# Autodesk Inventor assembly: Car_Assemblage_Etudiant_2024
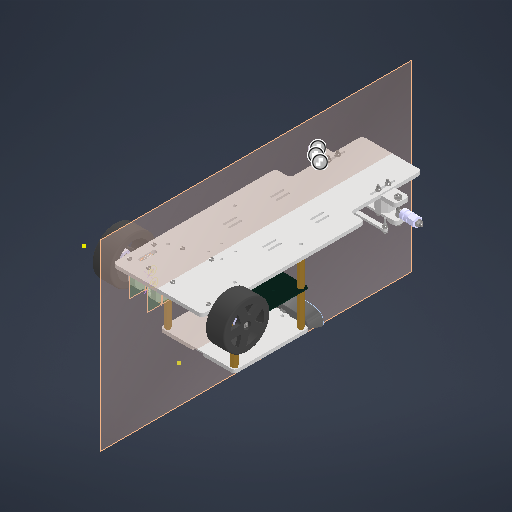
[picture p0: Inventor's stored thumbnail of the model, 512x512]
Saved by Autodesk Inventor 2027.1 (Build 311270010, 270A)
## iProperties
Created: 2023-10-18
Part Number: Car_Assemblage_Etudiant_2024
Document SubType Name: Assembly
Designer: baince
Mass: 835.359 g
Surface Area: 2295.89 cm^2
Volume: 721.463 cm^3
Density: 1.15787 g/cm^3
Author: baince
## Documents named in this file (38)
- C:\Users\thiag\Documents\ENSTA-1\Ateliers\CAO Inventor Etudiant\Car_Assemblage_Etudiant_2024.iam
- C:\Users\thiag\Documents\ENSTA-1\Ateliers\CAO Inventor Etudiant\chassis.ipt
- C:\Users\thiag\Documents\ENSTA-1\Ateliers\CAO Inventor Etudiant\support_avant.ipt
- C:\Users\thiag\Documents\ENSTA-1\Ateliers\CAO Inventor Etudiant\support_arriere_gauche.ipt
- C:\Users\thiag\Documents\ENSTA-1\Ateliers\CAO Inventor Etudiant\moteur_brushless.ipt
- C:\Users\thiag\Documents\ENSTA-1\Ateliers\CAO Inventor Etudiant\adaptateur roue.ipt
- C:\Users\thiag\Documents\ENSTA-1\Ateliers\CAO Inventor Etudiant\adaptateur_brushless.ipt
- C:\Users\thiag\Documents\ENSTA-1\Ateliers\CAO Inventor Etudiant\roue.ipt
- C:\Users\thiag\Documents\ENSTA-1\Ateliers\CAO Inventor Etudiant\biellette_servo_moteur.ipt
- C:\Users\thiag\Documents\ENSTA-1\Ateliers\CAO Inventor Etudiant\support_servo_moteur.ipt
- C:\Users\thiag\Documents\ENSTA-1\Ateliers\CAO Inventor Etudiant\SUPPORT_MOTEUR_BRUSHLESS2.IPT
- C:\Users\thiag\Documents\ENSTA-1\Ateliers\CAO Inventor Etudiant\corps_servo_moteur.ipt
- C:\Users\thiag\Documents\ENSTA-1\Ateliers\CAO Inventor Etudiant\batterie.ipt
- C:\Users\thiag\Documents\ENSTA-1\Ateliers\CAO Inventor Etudiant\roulement_6_19.ipt
- C:\Users\thiag\Documents\ENSTA-1\Ateliers\CAO Inventor Etudiant\pignon_15_dents.ipt
- C:\Users\thiag\Documents\ENSTA-1\Ateliers\CAO Inventor Etudiant\pignon_32_dents.ipt
- C:\Users\thiag\Documents\ENSTA-1\Ateliers\CAO Inventor Etudiant\axe_taraude_m4.ipt
- C:\Users\thiag\Documents\ENSTA-1\Ateliers\CAO Inventor Etudiant\roulement_4_13.ipt
- C:\Users\thiag\Documents\ENSTA-1\Ateliers\CAO Inventor Etudiant\ISO 4032 - M4 - ISO.ipt
- C:\Users\thiag\Documents\ENSTA-1\Ateliers\CAO Inventor Etudiant\ANSI B18.16.3M - Property Class 5 and 10 - Metric M3 x 0.5 Type de métal.ipt
- C:\Users\thiag\Documents\ENSTA-1\Ateliers\CAO Inventor Etudiant\ANSI B18.3.1M - M3x0,5 x 30(1).ipt
- C:\Users\thiag\Documents\ENSTA-1\Ateliers\CAO Inventor Etudiant\ISO 4762 - M4 x 30ISO.ipt
- C:\Users\thiag\Documents\ENSTA-1\Ateliers\CAO Inventor Etudiant\ISO 7089 - 4 - 140 HV(1).ipt
- C:\Users\thiag\Documents\ENSTA-1\Ateliers\CAO Inventor Etudiant\ISO 4762 - M4 x 35ISO.ipt
- C:\Users\thiag\Documents\ENSTA-1\Ateliers\CAO Inventor Etudiant\SKF623.ipt
- C:\Users\thiag\Documents\ENSTA-1\Ateliers\CAO Inventor Etudiant\ISO 7089 - 6 - 140 HV(1).ipt
- C:\Users\thiag\Documents\ENSTA-1\Ateliers\CAO Inventor Etudiant\ANSI B18.3.1M - M3x0,5 x 35(1).ipt
- C:\Users\thiag\Documents\ENSTA-1\Ateliers\CAO Inventor Etudiant\ISO 7089 - 3 - 140 HV(1).ipt
- C:\Users\thiag\Documents\ENSTA-1\Ateliers\CAO Inventor Etudiant\EN ISO 7045 - M3 x 14 - 4.8 - Z(2).ipt
- C:\Users\thiag\Documents\ENSTA-1\Ateliers\CAO Inventor Etudiant\VisM3-16.ipt
- C:\Users\thiag\Documents\ENSTA-1\Ateliers\CAO Inventor Etudiant\support_avant_MIR2.ipt
- C:\Users\thiag\Documents\ENSTA-1\Ateliers\CAO Inventor Etudiant\ESSIEU_ARRIERE.IPT
- C:\Users\thiag\Documents\ENSTA-1\Ateliers\CAO Inventor Etudiant\barre_direction.ipt
- C:\Users\thiag\Documents\ENSTA-1\Ateliers\CAO Inventor Etudiant\pcb_assembly.iam
- C:\Users\thiag\Documents\ENSTA-1\Ateliers\CAO Inventor Etudiant\sensors_haut.iam
- C:\Users\thiag\Documents\ENSTA-1\Ateliers\Seila\support_arriere_droite.ipt
- support_arriere_droite.ipt
- C:\Users\thiag\Documents\ENSTA-1\Ateliers\Seila\support_arriere_gauche_2.ipt
## Components (122 placed, 36 different names)
1. chassis:1 — Mate:1, Mate:5, Mate:19, Flush:1, Flush:2, Mate:21, Mate:22, Mate:23, Mate:26, Mate:27, Mate:28, Mate:66, Mate:68, Mate:70, Mate:72, Insert:57, Insert:58, Insert:59, Insert:60, Insert:61, Insert:62, Insert:63, Insert:64, Mate:74, Mate:75, Mate:80, Mate:102, Mate:103, Mate:104, Mate:118, Mate:120
2. ESSIEU ARRIERE:1 — Mate:115
3. support_avant:1 — Mate:1, Mate:3, Mate:4, Mate:5, Mate:7, Insert:30, Insert:84, Mate:87, Mate:89
4. moteur_brushless:1 — Mate:29, Mate:30, Mate:31, Insert:12
5. adaptateur roue:1 — Mate:43, Mate:44, Mate:45, Insert:18
6. adaptateur_brushless:1 — Mate:29, Mate:30, Mate:31, Mate:32, Mate:33, Mate:34, Insert:77, Insert:78, Insert:79, Insert:80
7. roue:1 — Mate:42, Mate:46, Mate:47, Insert:39
8. roue:2 — Mate:41, Mate:48, Mate:49, Insert:41
9. roue:3 — Mate:40, Mate:50, Mate:51, Insert:37
10. roue:4 — Mate:43, Mate:44, Mate:45, Insert:35
11. support_arriere_gauche:2 — Mate:21, Mate:22, Mate:23, Mate:36, Mate:38, Insert:65, Insert:69
12. biellette_servo_moteur:1 — Mate:15, Mate:16, Mate:101, Mate:116, Rotation:1
13. support_servo_moteur:1 — Mate:3, Mate:4, Mate:7, Mate:12, Mate:13, Mate:14, Insert:43, Insert:45, Insert:47, Insert:49, Angle:4
14. SUPPORT_MOTEUR_BRUSHLESS2:1 — Mate:26, Mate:27, Mate:28, Mate:32, Mate:33, Mate:34, Insert:66, Insert:70, Insert:73, Insert:74, Insert:75, Insert:76
15. corps_servo_moteur:1 — Mate:12, Mate:13, Mate:14, Mate:15, Mate:16
16. batterie:1 — Mate:19, Flush:1, Flush:2
17. roulement_6_19:1 — Insert:27, Mate:117
18. roulement_6_19:2 — Mate:36, Mate:38
19. adaptateur roue:2 — Mate:42, Mate:46, Mate:47
20. adaptateur roue:3 — Mate:41, Mate:48, Mate:49, Mate:115
21. adaptateur roue:4 — Mate:40, Mate:50, Mate:51, Insert:19
22. pignon_15_dents:1 — Insert:12, Tangent:1
23. pignon_32_dents:1 — Tangent:2
24. axe_taraude_m4:1 — Insert:25, Mate:63
25. roulement_4_13:1 — Insert:6, Mate:92, Mate:113
26. roulement_4_13:2 — Insert:3, Mate:114
27. roulement_4_13:3 — Insert:8, Mate:90
28. roulement_4_13:4 — Insert:10, Mate:109, Mate:110
29. ISO 4032 M4:1 — Insert:31
30. Ecrou hexagonal autofreiné - Acier Métrique Property Class 5 and 10 - Metric M3 x 0.5 Type de métal:1 — Insert:52
31. Vis à tête forgée - Métrique M3x0,5 x 30:1 — Insert:22, Mate:62
32. ISO 4762 M4 x 30:1 — Insert:2, Mate:111, Mate:112
33. ISO 4762 M4 x 30:2 — Insert:7, Mate:108, Mate:109
34. ISO 7089 4:1 — Insert:30, Insert:31
35. ISO 4762 M4 x 35:1 — Insert:83
36. ISO 4762 M4 x 35:2 — Insert:85
37. ISO 7089 4:2 — Insert:2, Insert:3
38. ISO 7089 4:3 — Insert:6, Insert:18
39. ISO 7089 4:4 — Insert:10, Insert:19
40. ISO 7089 4:5 — Insert:7, Insert:8
41. roulement_6_19:3 — Insert:25, Mate:81
42. SKF- roulements à une rangée de billes SKF623:1 — Insert:22, Insert:54
43. ISO 7089 6:1 — Insert:29, Mate:64, Mate:107
44. ISO 7089 6:2 — Insert:27
45. pignon_32_dents:2 — Mate:63, Mate:64, Tangent:1, Mate:81, Mate:107
46. pignon_15_dents:2 — Mate:62, Insert:29, Tangent:2
47. ISO 4032 M4:2 — Insert:32
48. ISO 4032 M4:3 — Insert:34
49. ISO 4032 M4:4 — Insert:36
50. ISO 4032 M4:5 — Insert:38
51. ISO 4032 M4:6 — Insert:40
52. ISO 7089 4:6 — Insert:34, Insert:35
53. ISO 7089 4:7 — Insert:36, Insert:37
54. ISO 7089 4:8 — Insert:38, Insert:39
55. ISO 7089 4:9 — Insert:40, Insert:41
56. ISO 7089 4:10 — Insert:32, Insert:96
57. Vis à tête forgée - Métrique M3x0,5 x 35:1 — Insert:42, Mate:69
58. Vis à tête forgée - Métrique M3x0,5 x 35:2 — Insert:44, Mate:71
59. Vis à tête forgée - Métrique M3x0,5 x 35:3 — Insert:48, Mate:65, Mate:76
60. Vis à tête forgée - Métrique M3x0,5 x 35:4 — Insert:46, Mate:67, Mate:79
61. Ecrou hexagonal autofreiné - Acier Métrique Property Class 5 and 10 - Metric M3 x 0.5 Type de métal:2 — Insert:50
62. Ecrou hexagonal autofreiné - Acier Métrique Property Class 5 and 10 - Metric M3 x 0.5 Type de métal:3 — Insert:51
63. Ecrou hexagonal autofreiné - Acier Métrique Property Class 5 and 10 - Metric M3 x 0.5 Type de métal:4 — Insert:53
64. ISO 7089 3:1 — Insert:44, Insert:45
65. ISO 7089 3:2 — Insert:46, Insert:47
66. ISO 7089 3:3 — Insert:52, Mate:71, Mate:72
67. ISO 7089 3:4 — Insert:53, Mate:65, Mate:66
68. ISO 7089 3:5 — Insert:48, Insert:49
69. ISO 7089 3:6 — Insert:54, Insert:55
70. ISO 7089 3:7 — Insert:50, Mate:69, Mate:70
71. ISO 7089 3:8 — Insert:42, Insert:43
72. ISO 7089 3:9 — Insert:51, Mate:67, Mate:68
73. ISO 7089 3:10 — Insert:55, Insert:56
74. ISO 7089 3:11 — Insert:56
75. NF EN ISO 7045 - Z M3 x 14 - 4.8 - Z:1 — Insert:60
76. NF EN ISO 7045 - Z M3 x 14 - 4.8 - Z:2 — Insert:59
77. NF EN ISO 7045 - Z M3 x 14 - 4.8 - Z:3 — Insert:58
78. NF EN ISO 7045 - Z M3 x 14 - 4.8 - Z:4 — Insert:57
79. NF EN ISO 7045 - Z M3 x 14 - 4.8 - Z:5 — Insert:61, Mate:123
80. NF EN ISO 7045 - Z M3 x 14 - 4.8 - Z:6 — Insert:62, Mate:119
81. NF EN ISO 7045 - Z M3 x 14 - 4.8 - Z:7 — Insert:63, Mate:122
82. NF EN ISO 7045 - Z M3 x 14 - 4.8 - Z:8 — Insert:64, Mate:121
83. Ecrou hexagonal autofreiné - Acier Métrique Property Class 5 and 10 - Metric M3 x 0.5 Type de métal:5 — Insert:65
84. Ecrou hexagonal autofreiné - Acier Métrique Property Class 5 and 10 - Metric M3 x 0.5 Type de métal:6
85. Ecrou hexagonal autofreiné - Acier Métrique Property Class 5 and 10 - Metric M3 x 0.5 Type de métal:7
86. Ecrou hexagonal autofreiné - Acier Métrique Property Class 5 and 10 - Metric M3 x 0.5 Type de métal:8 — Insert:66
87. Ecrou hexagonal autofreiné - Acier Métrique Property Class 5 and 10 - Metric M3 x 0.5 Type de métal:9 — Insert:75
88. Ecrou hexagonal autofreiné - Acier Métrique Property Class 5 and 10 - Metric M3 x 0.5 Type de métal:10 — Insert:69
89. Ecrou hexagonal autofreiné - Acier Métrique Property Class 5 and 10 - Metric M3 x 0.5 Type de métal:11 — Insert:70
90. Ecrou hexagonal autofreiné - Acier Métrique Property Class 5 and 10 - Metric M3 x 0.5 Type de métal:12 — Insert:73
91. Ecrou hexagonal autofreiné - Acier Métrique Property Class 5 and 10 - Metric M3 x 0.5 Type de métal:13
92. Ecrou hexagonal autofreiné - Acier Métrique Property Class 5 and 10 - Metric M3 x 0.5 Type de métal:14
93. Ecrou hexagonal autofreiné - Acier Métrique Property Class 5 and 10 - Metric M3 x 0.5 Type de métal:15 — Insert:74
94. Ecrou hexagonal autofreiné - Acier Métrique Property Class 5 and 10 - Metric M3 x 0.5 Type de métal:16 — Insert:76
95. NF EN ISO 7045 - Z M3 x 14 - 4.8 - Z:9 — Insert:77
96. NF EN ISO 7045 - Z M3 x 14 - 4.8 - Z:10 — Insert:78
97. NF EN ISO 7045 - Z M3 x 14 - 4.8 - Z:11 — Insert:80
98. NF EN ISO 7045 - Z M3 x 14 - 4.8 - Z:12 — Insert:79
99. VisM3-16:1 — Insert:88, Mate:126, Mate:127
100. VisM3-16:2 — Insert:89, Mate:124, Mate:125
101. Ecrou hexagonal autofreiné - Acier Métrique Property Class 5 and 10 - Metric M3 x 0.5 Type de métal:17 — Insert:87, Mate:127
102. Ecrou hexagonal autofreiné - Acier Métrique Property Class 5 and 10 - Metric M3 x 0.5 Type de métal:18 — Mate:125
103. ISO 7089 3:13
104. ISO 7089 3:14 — Insert:87
105. ISO 7089 3:15 — Insert:89, Mate:128
106. ISO 7089 4:11 — Insert:83, Insert:84
107. ISO 7089 4:12 — Insert:85, Insert:95
108. ISO 7089 3:16 — Insert:88, Mate:99
109. support_avant_MIR2:1 — Mate:74, Mate:75, Mate:76, Insert:95, Mate:79, Mate:80, Insert:96, Mate:85, Mate:88
110. barre_direction:1 — Mate:99, Mate:101, Mate:116, Mate:124, Mate:126, Rotation:1, Angle:4, Mate:128
111. ISO 7089 4:13 — Mate:88
112. ISO 7089 4:14 — Mate:85
113. ISO 7089 4:15 — Mate:87
114. ISO 7089 4:16 — Mate:89
115. ISO 7089 4:17 — Mate:91, Mate:108, Mate:110
116. ISO 7089 4:18 — Mate:90, Mate:91
117. ISO 7089 4:19 — Mate:93, Mate:111, Mate:114
118. ISO 7089 4:20 — Mate:92, Mate:93, Mate:112, Mate:113
119. pcb_assembly:1 [sub-assembly] — Mate:102, Mate:103, Mate:104, Mate:105, Mate:106
120. sensors_haut:1 [sub-assembly] — Mate:105, Mate:106
121. support_arriere_droite:1 — Mate:117, Mate:118, Mate:119, Mate:123
122. support_arriere_gauche_2:1 — Mate:120, Mate:121, Mate:122
## Relationships (173: Mate 94, Insert 70, Angle 3, Flush 2, Tangent 2, CylindricalJoint 1, RelateRotation 1)
- Mate:1: chassis:1 ↔ support_avant:1
- Mate:3: support_avant:1 ↔ support_servo_moteur:1
- Mate:4: support_avant:1 ↔ support_servo_moteur:1
- Mate:5: chassis:1 ↔ support_avant:1
- Mate:7: support_avant:1 ↔ support_servo_moteur:1
- Mate:12: support_servo_moteur:1 ↔ corps_servo_moteur:1
- Mate:13: support_servo_moteur:1 ↔ corps_servo_moteur:1
- Mate:14: support_servo_moteur:1 ↔ corps_servo_moteur:1
- Mate:15: biellette_servo_moteur:1 ↔ corps_servo_moteur:1
- Mate:16: biellette_servo_moteur:1 ↔ corps_servo_moteur:1
- Mate:19: chassis:1 ↔ batterie:1
- Flush:1 (43 mm): chassis:1 ↔ batterie:1
- Flush:2 (95 mm): chassis:1 ↔ batterie:1
- Mate:21: chassis:1 ↔ support_arriere_gauche:2
- Mate:22: chassis:1 ↔ support_arriere_gauche:2
- Mate:23: chassis:1 ↔ support_arriere_gauche:2
- [CylindricalJoint]: ESSIEU ARRIERE:1 ↔ support_arriere_gauche:2
- Mate:26: chassis:1 ↔ SUPPORT_MOTEUR_BRUSHLESS2:1
- Mate:27: chassis:1 ↔ SUPPORT_MOTEUR_BRUSHLESS2:1
- Mate:28: chassis:1 ↔ SUPPORT_MOTEUR_BRUSHLESS2:1
- Mate:29: moteur_brushless:1 ↔ adaptateur_brushless:1
- Mate:30: moteur_brushless:1 ↔ adaptateur_brushless:1
- Mate:31: moteur_brushless:1 ↔ adaptateur_brushless:1
- Mate:32: adaptateur_brushless:1 ↔ SUPPORT_MOTEUR_BRUSHLESS2:1
- Mate:33: adaptateur_brushless:1 ↔ SUPPORT_MOTEUR_BRUSHLESS2:1
- Mate:34: adaptateur_brushless:1 ↔ SUPPORT_MOTEUR_BRUSHLESS2:1
- Mate:36: support_arriere_gauche:2 ↔ roulement_6_19:2
- Mate:38: support_arriere_gauche:2 ↔ roulement_6_19:2
- [Mate]: ESSIEU ARRIERE:1 ↔ roulement_6_19:2
- Mate:40: roue:3 ↔ adaptateur roue:4
- Mate:41: roue:2 ↔ adaptateur roue:3
- Mate:42: roue:1 ↔ adaptateur roue:2
- Mate:43: adaptateur roue:1 ↔ roue:4
- Mate:44: adaptateur roue:1 ↔ roue:4
- Mate:45: adaptateur roue:1 ↔ roue:4
- Mate:46: roue:1 ↔ adaptateur roue:2
- Mate:47: roue:1 ↔ adaptateur roue:2
- Mate:48: roue:2 ↔ adaptateur roue:3
- Mate:49: roue:2 ↔ adaptateur roue:3
- Mate:50: roue:3 ↔ adaptateur roue:4
- Mate:51: roue:3 ↔ adaptateur roue:4
- [Mate]: ESSIEU ARRIERE:1 ↔ adaptateur roue:3
- [Angle] (0 deg): ESSIEU ARRIERE:1 ↔ adaptateur roue:3
- [Insert]: ESSIEU ARRIERE:1 ↔ adaptateur roue:2
- [Angle] (0 deg): ESSIEU ARRIERE:1 ↔ adaptateur roue:2
- Insert:2: ISO 4762 M4 x 30:1 ↔ ISO 7089 4:2
- Insert:3: roulement_4_13:2 ↔ ISO 7089 4:2
- Insert:6: roulement_4_13:1 ↔ ISO 7089 4:3
- Insert:7: ISO 4762 M4 x 30:2 ↔ ISO 7089 4:5
- Insert:8: roulement_4_13:3 ↔ ISO 7089 4:5
- Insert:10: roulement_4_13:4 ↔ ISO 7089 4:4
- Insert:12: moteur_brushless:1 ↔ pignon_15_dents:1
- Insert:18: adaptateur roue:1 ↔ ISO 7089 4:3
- Insert:19: adaptateur roue:4 ↔ ISO 7089 4:4
- Insert:22: Vis à tête forgée - Métrique M3x0,5 x 30:1 ↔ SKF- roulements à une rangée de billes SKF623:1
- Insert:25: axe_taraude_m4:1 ↔ roulement_6_19:3
- [Insert]: ESSIEU ARRIERE:1 ↔ pignon_32_dents:1
- [Mate]: ESSIEU ARRIERE:1 ↔ pignon_32_dents:1
- Insert:27: roulement_6_19:1 ↔ ISO 7089 6:2
- Mate:62: Vis à tête forgée - Métrique M3x0,5 x 30:1 ↔ pignon_15_dents:2
- Insert:29: ISO 7089 6:1 ↔ pignon_15_dents:2
- Mate:63: axe_taraude_m4:1 ↔ pignon_32_dents:2
- Mate:64: ISO 7089 6:1 ↔ pignon_32_dents:2
- Tangent:1: pignon_15_dents:1 ↔ pignon_32_dents:2
- Tangent:2: pignon_32_dents:1 ↔ pignon_15_dents:2
- Insert:30: support_avant:1 ↔ ISO 7089 4:1
- Insert:31: ISO 4032 M4:1 ↔ ISO 7089 4:1
- Insert:32: ISO 4032 M4:2 ↔ ISO 7089 4:10
- Insert:34: ISO 4032 M4:3 ↔ ISO 7089 4:6
- Insert:35: roue:4 ↔ ISO 7089 4:6
- Insert:36: ISO 4032 M4:4 ↔ ISO 7089 4:7
- Insert:37: roue:3 ↔ ISO 7089 4:7
- Insert:38: ISO 4032 M4:5 ↔ ISO 7089 4:8
- Insert:39: roue:1 ↔ ISO 7089 4:8
- Insert:40: ISO 4032 M4:6 ↔ ISO 7089 4:9
- Insert:41: roue:2 ↔ ISO 7089 4:9
- Insert:42: Vis à tête forgée - Métrique M3x0,5 x 35:1 ↔ ISO 7089 3:8
- Insert:43: support_servo_moteur:1 ↔ ISO 7089 3:8
- Insert:44: Vis à tête forgée - Métrique M3x0,5 x 35:2 ↔ ISO 7089 3:1
- Insert:45: support_servo_moteur:1 ↔ ISO 7089 3:1
- Insert:46: Vis à tête forgée - Métrique M3x0,5 x 35:4 ↔ ISO 7089 3:2
- Insert:47: support_servo_moteur:1 ↔ ISO 7089 3:2
- Insert:48: Vis à tête forgée - Métrique M3x0,5 x 35:3 ↔ ISO 7089 3:5
- Insert:49: support_servo_moteur:1 ↔ ISO 7089 3:5
- Insert:50: Ecrou hexagonal autofreiné - Acier Métrique Property Class 5 and 10 - Metric M3 x 0.5 Type de métal:2 ↔ ISO 7089 3:7
- Insert:51: Ecrou hexagonal autofreiné - Acier Métrique Property Class 5 and 10 - Metric M3 x 0.5 Type de métal:3 ↔ ISO 7089 3:9
- Insert:52: Ecrou hexagonal autofreiné - Acier Métrique Property Class 5 and 10 - Metric M3 x 0.5 Type de métal:1 ↔ ISO 7089 3:3
- Insert:53: Ecrou hexagonal autofreiné - Acier Métrique Property Class 5 and 10 - Metric M3 x 0.5 Type de métal:4 ↔ ISO 7089 3:4
- Mate:65: Vis à tête forgée - Métrique M3x0,5 x 35:3 ↔ ISO 7089 3:4
- Mate:66: chassis:1 ↔ ISO 7089 3:4
- Mate:67: Vis à tête forgée - Métrique M3x0,5 x 35:4 ↔ ISO 7089 3:9
- Mate:68: chassis:1 ↔ ISO 7089 3:9
- Mate:69: Vis à tête forgée - Métrique M3x0,5 x 35:1 ↔ ISO 7089 3:7
- Mate:70: chassis:1 ↔ ISO 7089 3:7
- Mate:71: Vis à tête forgée - Métrique M3x0,5 x 35:2 ↔ ISO 7089 3:3
- Mate:72: chassis:1 ↔ ISO 7089 3:3
- Insert:54: SKF- roulements à une rangée de billes SKF623:1 ↔ ISO 7089 3:6
- Insert:55: ISO 7089 3:6 ↔ ISO 7089 3:10
- Insert:56: ISO 7089 3:10 ↔ ISO 7089 3:11
- Insert:57: chassis:1 ↔ NF EN ISO 7045 - Z M3 x 14 - 4.8 - Z:4
- Insert:58: chassis:1 ↔ NF EN ISO 7045 - Z M3 x 14 - 4.8 - Z:3
- Insert:59: chassis:1 ↔ NF EN ISO 7045 - Z M3 x 14 - 4.8 - Z:2
- Insert:60: chassis:1 ↔ NF EN ISO 7045 - Z M3 x 14 - 4.8 - Z:1
- Insert:61: chassis:1 ↔ NF EN ISO 7045 - Z M3 x 14 - 4.8 - Z:5
- Insert:62: chassis:1 ↔ NF EN ISO 7045 - Z M3 x 14 - 4.8 - Z:6
- Insert:63: chassis:1 ↔ NF EN ISO 7045 - Z M3 x 14 - 4.8 - Z:7
- Insert:64: chassis:1 ↔ NF EN ISO 7045 - Z M3 x 14 - 4.8 - Z:8
- Insert:65: support_arriere_gauche:2 ↔ Ecrou hexagonal autofreiné - Acier Métrique Property Class 5 and 10 - Metric M3 x 0.5 Type de métal:5
- Insert:66: SUPPORT_MOTEUR_BRUSHLESS2:1 ↔ Ecrou hexagonal autofreiné - Acier Métrique Property Class 5 and 10 - Metric M3 x 0.5 Type de métal:8
- Insert:69: support_arriere_gauche:2 ↔ Ecrou hexagonal autofreiné - Acier Métrique Property Class 5 and 10 - Metric M3 x 0.5 Type de métal:10
- Insert:70: SUPPORT_MOTEUR_BRUSHLESS2:1 ↔ Ecrou hexagonal autofreiné - Acier Métrique Property Class 5 and 10 - Metric M3 x 0.5 Type de métal:11
- Insert:73: SUPPORT_MOTEUR_BRUSHLESS2:1 ↔ Ecrou hexagonal autofreiné - Acier Métrique Property Class 5 and 10 - Metric M3 x 0.5 Type de métal:12
- Insert:74: SUPPORT_MOTEUR_BRUSHLESS2:1 ↔ Ecrou hexagonal autofreiné - Acier Métrique Property Class 5 and 10 - Metric M3 x 0.5 Type de métal:15
- Insert:75: SUPPORT_MOTEUR_BRUSHLESS2:1 ↔ Ecrou hexagonal autofreiné - Acier Métrique Property Class 5 and 10 - Metric M3 x 0.5 Type de métal:9
- Insert:76: SUPPORT_MOTEUR_BRUSHLESS2:1 ↔ Ecrou hexagonal autofreiné - Acier Métrique Property Class 5 and 10 - Metric M3 x 0.5 Type de métal:16
- Insert:77: adaptateur_brushless:1 ↔ NF EN ISO 7045 - Z M3 x 14 - 4.8 - Z:9
- Insert:78: adaptateur_brushless:1 ↔ NF EN ISO 7045 - Z M3 x 14 - 4.8 - Z:10
- Insert:79: adaptateur_brushless:1 ↔ NF EN ISO 7045 - Z M3 x 14 - 4.8 - Z:12
- Insert:80: adaptateur_brushless:1 ↔ NF EN ISO 7045 - Z M3 x 14 - 4.8 - Z:11
- [Insert]: Ecrou hexagonal autofreiné - Acier Métrique Property Class 5 and 10 - Metric M3 x 0.5 Type de métal:18 ↔ ISO 7089 3:13
- Insert:83: ISO 4762 M4 x 35:1 ↔ ISO 7089 4:11
- Insert:84: support_avant:1 ↔ ISO 7089 4:11
- Insert:85: ISO 4762 M4 x 35:2 ↔ ISO 7089 4:12
- Insert:87: Ecrou hexagonal autofreiné - Acier Métrique Property Class 5 and 10 - Metric M3 x 0.5 Type de métal:17 ↔ ISO 7089 3:14
- Insert:88: VisM3-16:1 ↔ ISO 7089 3:16
- Insert:89: VisM3-16:2 ↔ ISO 7089 3:15
- Mate:74: chassis:1 ↔ support_avant_MIR2:1
- Mate:75: chassis:1 ↔ support_avant_MIR2:1
- Mate:76: Vis à tête forgée - Métrique M3x0,5 x 35:3 ↔ support_avant_MIR2:1
- Insert:95: ISO 7089 4:12 ↔ support_avant_MIR2:1
- Mate:79: Vis à tête forgée - Métrique M3x0,5 x 35:4 ↔ support_avant_MIR2:1
- Mate:80 (-40 mm): chassis:1 ↔ support_avant_MIR2:1
- Insert:96: ISO 7089 4:10 ↔ support_avant_MIR2:1
- Mate:81: roulement_6_19:3 ↔ pignon_32_dents:2
- Mate:85: support_avant_MIR2:1 ↔ ISO 7089 4:14
- Mate:87: support_avant:1 ↔ ISO 7089 4:15
- Mate:88: support_avant_MIR2:1 ↔ ISO 7089 4:13
- Mate:89: support_avant:1 ↔ ISO 7089 4:16
- Mate:90: roulement_4_13:3 ↔ ISO 7089 4:18
- Mate:91: ISO 7089 4:17 ↔ ISO 7089 4:18
- Mate:92: roulement_4_13:1 ↔ ISO 7089 4:20
- Mate:93: ISO 7089 4:19 ↔ ISO 7089 4:20
- Mate:99: ISO 7089 3:16 ↔ barre_direction:1
- Mate:101: biellette_servo_moteur:1 ↔ barre_direction:1
- Mate:102: chassis:1 ↔ pcb_assembly:1
- Mate:103: chassis:1 ↔ pcb_assembly:1
- Mate:104: chassis:1 ↔ pcb_assembly:1
- Mate:105: pcb_assembly:1 ↔ sensors_haut:1
- Mate:106: pcb_assembly:1 ↔ sensors_haut:1
- Mate:107: ISO 7089 6:1 ↔ pignon_32_dents:2
- Mate:108: ISO 4762 M4 x 30:2 ↔ ISO 7089 4:17
- Mate:109: roulement_4_13:4 ↔ ISO 4762 M4 x 30:2
- Mate:110: roulement_4_13:4 ↔ ISO 7089 4:17
- Mate:111: ISO 4762 M4 x 30:1 ↔ ISO 7089 4:19
- Mate:112: ISO 4762 M4 x 30:1 ↔ ISO 7089 4:20
- Mate:113: roulement_4_13:1 ↔ ISO 7089 4:20
- Mate:114: roulement_4_13:2 ↔ ISO 7089 4:19
- Mate:115: ESSIEU ARRIERE:1 ↔ adaptateur roue:3
- Mate:116: biellette_servo_moteur:1 ↔ barre_direction:1
- Mate:117: roulement_6_19:1 ↔ support_arriere_droite:1
- Mate:118: chassis:1 ↔ support_arriere_droite:1
- Mate:119: NF EN ISO 7045 - Z M3 x 14 - 4.8 - Z:6 ↔ support_arriere_droite:1
- Mate:120: chassis:1 ↔ support_arriere_gauche_2:1
- Mate:121: NF EN ISO 7045 - Z M3 x 14 - 4.8 - Z:8 ↔ support_arriere_gauche_2:1
- Mate:122: NF EN ISO 7045 - Z M3 x 14 - 4.8 - Z:7 ↔ support_arriere_gauche_2:1
- Mate:123: NF EN ISO 7045 - Z M3 x 14 - 4.8 - Z:5 ↔ support_arriere_droite:1
- Mate:124: VisM3-16:2 ↔ barre_direction:1
- Mate:125: VisM3-16:2 ↔ Ecrou hexagonal autofreiné - Acier Métrique Property Class 5 and 10 - Metric M3 x 0.5 Type de métal:18
- Mate:126: VisM3-16:1 ↔ barre_direction:1
- Mate:127: VisM3-16:1 ↔ Ecrou hexagonal autofreiné - Acier Métrique Property Class 5 and 10 - Metric M3 x 0.5 Type de métal:17
- Rotation:1 [RelateRotation]: biellette_servo_moteur:1 ↔ barre_direction:1
- Angle:4 (90 deg): support_servo_moteur:1 ↔ barre_direction:1
- Mate:128: ISO 7089 3:15 ↔ barre_direction:1
## Named parameters: d185_d147 = 0 mm
